# Autodesk Inventor assembly: MECANISMO DE COMPACTADO
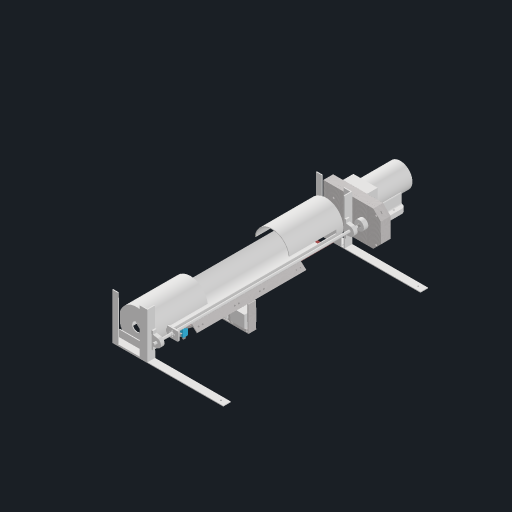
[picture p0: Inventor's stored thumbnail of the model, 512x512]
Saved by Autodesk Inventor 2024.3 (Build 283343000, 343)
## iProperties
Created: 2024-05-26
Part Number: MECANISMO DE COMPACTADO
Document SubType Name: Assembly
Designer: Jhuliams
Author: Jhuliams
## Documents named in this file (32)
- C:\Users\Niler\OneDrive\Escritorio\RECICLADOR\RECICLADOR_MODELO_3D\MECANISMO DE COMPACTADO\MECANISMO DE COMPACTADO.iam
- C:\Users\Niler\OneDrive\Escritorio\RECICLADOR\RECICLADOR_MODELO_3D\MECANISMO DE COMPACTADO\GUIA_DE_OBJETO.ipt
- C:\Users\Niler\OneDrive\Escritorio\RECICLADOR\RECICLADOR_MODELO_3D\MECANISMO DE COMPACTADO\TAPA QUE DESPLAZA CON TORNILLOS.ipt
- C:\Users\Niler\OneDrive\Escritorio\RECICLADOR\RECICLADOR_MODELO_3D\MECANISMO DE COMPACTADO\TUERCA DE HUSILLO.ipt
- C:\Users\Niler\OneDrive\Escritorio\RECICLADOR\RECICLADOR_MODELO_3D\MECANISMO DE COMPACTADO\TORNILLO DEPOTENCIA.ipt
- C:\Users\Niler\OneDrive\Escritorio\RECICLADOR\RECICLADOR_MODELO_3D\MECANISMO DE COMPACTADO\ACOPLE HELICOIDAL.ipt
- C:\Users\Niler\OneDrive\Escritorio\RECICLADOR\RECICLADOR_MODELO_3D\MECANISMO DE COMPACTADO\RODAMIENTO DE TORNILLO.ipt
- C:\Users\Niler\OneDrive\Escritorio\RECICLADOR\RECICLADOR_MODELO_3D\MECANISMO DE COMPACTADO\PLETINA PARA GUIA CILINDRICA.ipt
- C:\Users\Niler\OneDrive\Escritorio\RECICLADOR\RECICLADOR_MODELO_3D\MECANISMO DE COMPACTADO\SOPORTE LATERAL DE GUIA CILINDRICA.ipt
- C:\Users\Niler\OneDrive\Escritorio\RECICLADOR\RECICLADOR_MODELO_3D\MECANISMO DE COMPACTADO\SOPORTE LATERAL DE GUIA CILINDRICA_MIR.ipt
- C:\Users\Niler\OneDrive\Escritorio\RECICLADOR\RECICLADOR_MODELO_3D\MECANISMO DE COMPACTADO\RODAMIENTO DE TORNILLO_MIR.ipt
- C:\Users\Niler\OneDrive\Escritorio\RECICLADOR\RECICLADOR_MODELO_3D\MECANISMO DE COMPACTADO\SOPORTE LATERAL DE GUIA CILINDRICA_MIR1.ipt
- C:\Users\Niler\OneDrive\Escritorio\RECICLADOR\RECICLADOR_MODELO_3D\MECANISMO DE COMPACTADO\RODAMIENTO DE TORNILLO_MIR1.ipt
- C:\Users\Niler\OneDrive\Escritorio\RECICLADOR\RECICLADOR_MODELO_3D\MECANISMO DE COMPACTADO\SOPORTE LATERAL DE GUIA CILINDRICA_MIR2.ipt
- C:\Users\Niler\OneDrive\Escritorio\RECICLADOR\RECICLADOR_MODELO_3D\MECANISMO DE COMPACTADO\RODAMIENTO DE TORNILLO_MIR_MIR.ipt
- C:\Users\Niler\OneDrive\Escritorio\RECICLADOR\RECICLADOR_MODELO_3D\MECANISMO DE COMPACTADO\SOPORTE LATERAL DE GUIA CILINDRICA_MIR1_MIR.ipt
- C:\Users\Niler\OneDrive\Escritorio\RECICLADOR\RECICLADOR_MODELO_3D\MECANISMO DE COMPACTADO\ACOPLE HELICOIDAL_MIR.ipt
- C:\Users\Niler\OneDrive\Escritorio\RECICLADOR\RECICLADOR_MODELO_3D\CAJA_ENGRANAJES\VERSION_3\CAJA_ENGRANAJES_COMPLETA_V3.iam
- C:\Users\Niler\OneDrive\Escritorio\RECICLADOR\RECICLADOR_MODELO_3D\NUEVA_PARTE_MECANISMO_COMPACTADO\CANALETA_MOVIL.ipt
- C:\Users\Niler\OneDrive\Escritorio\RECICLADOR\RECICLADOR_MODELO_3D\NUEVA_PARTE_MECANISMO_COMPACTADO\APORYO_CANALETA_,MOVIL.ipt
- C:\Users\Niler\OneDrive\Escritorio\RECICLADOR\RECICLADOR_MODELO_3D\NUEVA_PARTE_MECANISMO_COMPACTADO\PLENTINA_CANALETA_MOVIL.ipt
- C:\Users\Niler\OneDrive\Escritorio\RECICLADOR\RECICLADOR_MODELO_3D\NUEVA_PARTE_MECANISMO_COMPACTADO\APORYO_CANALETA_,MOVIL_P2.ipt
- C:\Users\Niler\OneDrive\Escritorio\RECICLADOR\RECICLADOR_MODELO_3D\NUEVA_PARTE_MECANISMO_COMPACTADO\CREMALLERA_CANALETA_MOVIL.ipt
- C:\Users\Niler\OneDrive\Escritorio\RECICLADOR\RECICLADOR_MODELO_3D\NUEVA_PARTE_MECANISMO_COMPACTADO\SOPORTE_METAL_PAP.ipt
- C:\Users\Niler\OneDrive\Escritorio\RECICLADOR\RECICLADOR_MODELO_3D\MECANISMO DE COMPACTADO\PINON DE TAPA PRINCIPAL.ipt
- C:\Users\Niler\OneDrive\Escritorio\RECICLADOR\RECICLADOR_MODELO_3D\MECANISMO DE COMPACTADO\NEMA 17 PARA TAPA PRINCIPAL.ipt
- C:\Users\Niler\OneDrive\Escritorio\RECICLADOR\RECICLADOR_MODELO_3D\MECANISMO DE COMPACTADO\ACOPLE_NEMA_PUERTA.ipt
- C:\Users\Niler\OneDrive\Escritorio\RECICLADOR\RECICLADOR_MODELO_3D\VERSION_3_COMPLETA\FIN_DE_CARRERA.ipt
- C:\Users\Niler\OneDrive\Escritorio\RECICLADOR\RECICLADOR_MODELO_3D\NUEVA_PARTE_MECANISMO_COMPACTADO\APORYO_CANALETA_,MOVIL_MIR.ipt
- C:\Users\Niler\OneDrive\Escritorio\RECICLADOR\RECICLADOR_MODELO_3D\VERSION_3_COMPLETA\FIN_DE_CARRERA_MIR.ipt
- C:\Users\Niler\OneDrive\Escritorio\RECICLADOR\RECICLADOR_MODELO_3D\NUEVA_PARTE_MECANISMO_COMPACTADO\SOPORTE_CANALETA_PRINCIPAL.ipt
- C:\Users\Niler\OneDrive\Escritorio\RECICLADOR\RECICLADOR_MODELO_3D\Spur Gear11.ipt
## Components (39 placed, 31 different names)
1. PLETINA PARA GUIA CILINDRICA:1 — Mate:22, Flush:3, Mate:24, Flush:4, Flush:7, Flush:13, Flush:15, Mate:37
2. GUIA_DE_OBJETO:1 — Mate:6, Mate:7, Mate:8, Flush:2, Mate:21, Tangent:1, Mate:29, Tangent:2, Mate:42, Flush:23, Mate:52, Flush:25, Flush:30
3. TORNILLO DEPOTENCIA:1 — Mate:9, Mate:16, Flush:1, Mate:23, Mate:27, Flush:12, Mate:38, Mate:39
4. TORNILLO DEPOTENCIA:2 — Mate:10, Mate:15, Flush:1, Mate:34, Mate:35
5. TAPA QUE DESPLAZA CON TORNILLOS:1 — Mate:6, Mate:7, Mate:8, Mate:9, Mate:10, Mate:17, Mate:18, Mate:19, Mate:20
6. TUERCA DE HUSILLO:1 — Mate:16, Mate:17, Mate:20
7. TUERCA DE HUSILLO:2 — Mate:15, Mate:18, Mate:19
8. SOPORTE LATERAL DE GUIA CILINDRICA:1 — Flush:2, Mate:21, Tangent:1, Mate:22, Flush:3
9. SOPORTE LATERAL DE GUIA CILINDRICA_MIR:1 — Mate:29, Tangent:2, Mate:31, Flush:8, Mate:80
10. RODAMIENTO DE TORNILLO:1 — Mate:23, Mate:25, Flush:6, Flush:12
11. SOPORTE LATERAL DE GUIA CILINDRICA:2 — Mate:24, Mate:25, Flush:4, Flush:6
12. RODAMIENTO DE TORNILLO_MIR:1 — Mate:26, Flush:5, Mate:27
13. SOPORTE LATERAL DE GUIA CILINDRICA_MIR1:1 — Mate:26, Flush:5, Mate:30, Flush:9, Flush:22
14. PLETINA PARA GUIA CILINDRICA:2 — Flush:7, Mate:30, Mate:31, Flush:8, Flush:9, Flush:13, Mate:36, Flush:14, Flush:22
15. RODAMIENTO DE TORNILLO_MIR1:1 — Flush:10, Mate:32, Mate:35
16. SOPORTE LATERAL DE GUIA CILINDRICA_MIR2:1 — Flush:10, Mate:32, Flush:15, Mate:37
17. RODAMIENTO DE TORNILLO_MIR_MIR:1 — Flush:11, Mate:33, Mate:34
18. SOPORTE LATERAL DE GUIA CILINDRICA_MIR1_MIR:1 — Flush:11, Mate:33, Mate:36, Flush:14
19. ACOPLE HELICOIDAL:1 — Mate:38, Mate:39, Mate:40
20. ACOPLE HELICOIDAL_MIR:1 — Mate:41
21. CAJA_ENGRANAJES_COMPLETA_V3:1 [sub-assembly] — Mate:40, Mate:41
22. CANALETA_MOVIL:1 — Mate:42, Flush:23, Mate:65, Flush:26, Flush:27
23. APORYO_CANALETA_,MOVIL:1 — Mate:44, Mate:45, Mate:48, Mate:49, Mate:50, Mate:52, Mate:74, Mate:75, Mate:76, Flush:30
24. PLENTINA_CANALETA_MOVIL:1 — Mate:49, Mate:50, Mate:56, Mate:57, Mate:58, Mate:62, Mate:63, Mate:64, Mate:66
25. PLENTINA_CANALETA_MOVIL:2 — Mate:44, Mate:45, Mate:48, Flush:25, Mate:53, Mate:54, Mate:55, Mate:59, Mate:60, Mate:61, Mate:67, Flush:28
26. APORYO_CANALETA_,MOVIL_P2:1 — Mate:53, Mate:54, Mate:55
27. APORYO_CANALETA_,MOVIL_P2:2 — Mate:59, Mate:60, Mate:61
28. APORYO_CANALETA_,MOVIL_P2:3 — Mate:56, Mate:57, Mate:58
29. APORYO_CANALETA_,MOVIL_P2:4 — Mate:62, Mate:63, Mate:64
30. CREMALLERA_CANALETA_MOVIL:1 — Mate:65, Flush:26, Flush:27, Rotation/Translation:1
31. SOPORTE_METAL_PAP:1 — Mate:66, Mate:67, Flush:28, Mate:72, Flush:29, Mate:73
32. PINON DE TAPA PRINCIPAL:1 — Rotation/Translation:1, Mate:81, Mate:82
33. NEMA 17 PARA TAPA PRINCIPAL:1 — Mate:81
34. ACOPLE_NEMA_PUERTA:1 — Mate:72, Flush:29, Mate:73
35. FIN_DE_CARRERA:1 — Mate:74, Mate:75, Mate:76
36. APORYO_CANALETA_,MOVIL_MIR:1 — Mate:77, Mate:78, Mate:79
37. FIN_DE_CARRERA_MIR:1 — Mate:77, Mate:78, Mate:79
38. SOPORTE_CANALETA_PRINCIPAL:1 — Mate:80
39. Spur Gear1:1 — Mate:82
## Relationships (95: Mate 68, Flush 23, Tangent 2, Angle 1, RelateRotateTranslate 1)
- Mate:6: GUIA_DE_OBJETO:1 ↔ TAPA QUE DESPLAZA CON TORNILLOS:1
- Mate:7 (1 mm): GUIA_DE_OBJETO:1 ↔ TAPA QUE DESPLAZA CON TORNILLOS:1
- Mate:8 (1 mm): GUIA_DE_OBJETO:1 ↔ TAPA QUE DESPLAZA CON TORNILLOS:1
- Mate:9: TORNILLO DEPOTENCIA:1 ↔ TAPA QUE DESPLAZA CON TORNILLOS:1
- Mate:10: TORNILLO DEPOTENCIA:2 ↔ TAPA QUE DESPLAZA CON TORNILLOS:1
- Mate:15: TORNILLO DEPOTENCIA:2 ↔ TUERCA DE HUSILLO:2
- Mate:16: TORNILLO DEPOTENCIA:1 ↔ TUERCA DE HUSILLO:1
- Mate:17: TAPA QUE DESPLAZA CON TORNILLOS:1 ↔ TUERCA DE HUSILLO:1
- Mate:18: TAPA QUE DESPLAZA CON TORNILLOS:1 ↔ TUERCA DE HUSILLO:2
- Mate:19: TAPA QUE DESPLAZA CON TORNILLOS:1 ↔ TUERCA DE HUSILLO:2
- Mate:20: TAPA QUE DESPLAZA CON TORNILLOS:1 ↔ TUERCA DE HUSILLO:1
- Flush:1: TORNILLO DEPOTENCIA:1 ↔ TORNILLO DEPOTENCIA:2
- Flush:2 (48.325 mm): GUIA_DE_OBJETO:1 ↔ SOPORTE LATERAL DE GUIA CILINDRICA:1
- Mate:21: GUIA_DE_OBJETO:1 ↔ SOPORTE LATERAL DE GUIA CILINDRICA:1
- Tangent:1 (-7.5 mm): GUIA_DE_OBJETO:1 ↔ SOPORTE LATERAL DE GUIA CILINDRICA:1
- Mate:22: PLETINA PARA GUIA CILINDRICA:1 ↔ SOPORTE LATERAL DE GUIA CILINDRICA:1
- Flush:3: PLETINA PARA GUIA CILINDRICA:1 ↔ SOPORTE LATERAL DE GUIA CILINDRICA:1
- Mate:23: TORNILLO DEPOTENCIA:1 ↔ RODAMIENTO DE TORNILLO:1
- Mate:24: PLETINA PARA GUIA CILINDRICA:1 ↔ SOPORTE LATERAL DE GUIA CILINDRICA:2
- Mate:25: RODAMIENTO DE TORNILLO:1 ↔ SOPORTE LATERAL DE GUIA CILINDRICA:2
- Flush:4: PLETINA PARA GUIA CILINDRICA:1 ↔ SOPORTE LATERAL DE GUIA CILINDRICA:2
- Mate:26: RODAMIENTO DE TORNILLO_MIR:1 ↔ SOPORTE LATERAL DE GUIA CILINDRICA_MIR1:1
- Flush:5: RODAMIENTO DE TORNILLO_MIR:1 ↔ SOPORTE LATERAL DE GUIA CILINDRICA_MIR1:1
- Mate:27: TORNILLO DEPOTENCIA:1 ↔ RODAMIENTO DE TORNILLO_MIR:1
- Flush:6: RODAMIENTO DE TORNILLO:1 ↔ SOPORTE LATERAL DE GUIA CILINDRICA:2
- Mate:29: GUIA_DE_OBJETO:1 ↔ SOPORTE LATERAL DE GUIA CILINDRICA_MIR:1
- Tangent:2 (-107.5 mm): GUIA_DE_OBJETO:1 ↔ SOPORTE LATERAL DE GUIA CILINDRICA_MIR:1
- Flush:7: PLETINA PARA GUIA CILINDRICA:1 ↔ PLETINA PARA GUIA CILINDRICA:2
- Mate:30: SOPORTE LATERAL DE GUIA CILINDRICA_MIR1:1 ↔ PLETINA PARA GUIA CILINDRICA:2
- Mate:31: SOPORTE LATERAL DE GUIA CILINDRICA_MIR:1 ↔ PLETINA PARA GUIA CILINDRICA:2
- Flush:8: SOPORTE LATERAL DE GUIA CILINDRICA_MIR:1 ↔ PLETINA PARA GUIA CILINDRICA:2
- Flush:9: SOPORTE LATERAL DE GUIA CILINDRICA_MIR1:1 ↔ PLETINA PARA GUIA CILINDRICA:2
- Flush:10: RODAMIENTO DE TORNILLO_MIR1:1 ↔ SOPORTE LATERAL DE GUIA CILINDRICA_MIR2:1
- Mate:32: RODAMIENTO DE TORNILLO_MIR1:1 ↔ SOPORTE LATERAL DE GUIA CILINDRICA_MIR2:1
- Flush:11: RODAMIENTO DE TORNILLO_MIR_MIR:1 ↔ SOPORTE LATERAL DE GUIA CILINDRICA_MIR1_MIR:1
- Mate:33: RODAMIENTO DE TORNILLO_MIR_MIR:1 ↔ SOPORTE LATERAL DE GUIA CILINDRICA_MIR1_MIR:1
- Flush:12 (10 mm): TORNILLO DEPOTENCIA:1 ↔ RODAMIENTO DE TORNILLO:1
- Flush:13: PLETINA PARA GUIA CILINDRICA:1 ↔ PLETINA PARA GUIA CILINDRICA:2
- Mate:34: TORNILLO DEPOTENCIA:2 ↔ RODAMIENTO DE TORNILLO_MIR_MIR:1
- Mate:35: TORNILLO DEPOTENCIA:2 ↔ RODAMIENTO DE TORNILLO_MIR1:1
- Mate:36: PLETINA PARA GUIA CILINDRICA:2 ↔ SOPORTE LATERAL DE GUIA CILINDRICA_MIR1_MIR:1
- Flush:14: PLETINA PARA GUIA CILINDRICA:2 ↔ SOPORTE LATERAL DE GUIA CILINDRICA_MIR1_MIR:1
- Flush:15: PLETINA PARA GUIA CILINDRICA:1 ↔ SOPORTE LATERAL DE GUIA CILINDRICA_MIR2:1
- Mate:37: PLETINA PARA GUIA CILINDRICA:1 ↔ SOPORTE LATERAL DE GUIA CILINDRICA_MIR2:1
- Mate:38 (-20 mm): TORNILLO DEPOTENCIA:1 ↔ ACOPLE HELICOIDAL:1
- Mate:39: TORNILLO DEPOTENCIA:1 ↔ ACOPLE HELICOIDAL:1
- Flush:22 (250 mm): SOPORTE LATERAL DE GUIA CILINDRICA_MIR1:1 ↔ PLETINA PARA GUIA CILINDRICA:2
- Mate:40: ACOPLE HELICOIDAL:1 ↔ CAJA_ENGRANAJES_COMPLETA_V3:1
- Mate:41: ACOPLE HELICOIDAL_MIR:1 ↔ CAJA_ENGRANAJES_COMPLETA_V3:1
- Mate:42: GUIA_DE_OBJETO:1 ↔ CANALETA_MOVIL:1
- Flush:23: GUIA_DE_OBJETO:1 ↔ CANALETA_MOVIL:1
- Mate:44: APORYO_CANALETA_,MOVIL:1 ↔ PLENTINA_CANALETA_MOVIL:2
- Mate:45: APORYO_CANALETA_,MOVIL:1 ↔ PLENTINA_CANALETA_MOVIL:2
- Mate:48: APORYO_CANALETA_,MOVIL:1 ↔ PLENTINA_CANALETA_MOVIL:2
- Mate:49: APORYO_CANALETA_,MOVIL:1 ↔ PLENTINA_CANALETA_MOVIL:1
- Mate:50: APORYO_CANALETA_,MOVIL:1 ↔ PLENTINA_CANALETA_MOVIL:1
- Mate:52: GUIA_DE_OBJETO:1 ↔ APORYO_CANALETA_,MOVIL:1
- Flush:25: GUIA_DE_OBJETO:1 ↔ PLENTINA_CANALETA_MOVIL:2
- Mate:53: PLENTINA_CANALETA_MOVIL:2 ↔ APORYO_CANALETA_,MOVIL_P2:1
- Mate:54: PLENTINA_CANALETA_MOVIL:2 ↔ APORYO_CANALETA_,MOVIL_P2:1
- Mate:55: PLENTINA_CANALETA_MOVIL:2 ↔ APORYO_CANALETA_,MOVIL_P2:1
- Mate:56: PLENTINA_CANALETA_MOVIL:1 ↔ APORYO_CANALETA_,MOVIL_P2:3
- Mate:57: PLENTINA_CANALETA_MOVIL:1 ↔ APORYO_CANALETA_,MOVIL_P2:3
- Mate:58: PLENTINA_CANALETA_MOVIL:1 ↔ APORYO_CANALETA_,MOVIL_P2:3
- Mate:59: PLENTINA_CANALETA_MOVIL:2 ↔ APORYO_CANALETA_,MOVIL_P2:2
- Mate:60: PLENTINA_CANALETA_MOVIL:2 ↔ APORYO_CANALETA_,MOVIL_P2:2
- Mate:61: PLENTINA_CANALETA_MOVIL:2 ↔ APORYO_CANALETA_,MOVIL_P2:2
- Mate:62: PLENTINA_CANALETA_MOVIL:1 ↔ APORYO_CANALETA_,MOVIL_P2:4
- Mate:63: PLENTINA_CANALETA_MOVIL:1 ↔ APORYO_CANALETA_,MOVIL_P2:4
- Mate:64: PLENTINA_CANALETA_MOVIL:1 ↔ APORYO_CANALETA_,MOVIL_P2:4
- Mate:65: CANALETA_MOVIL:1 ↔ CREMALLERA_CANALETA_MOVIL:1
- Flush:26: CANALETA_MOVIL:1 ↔ CREMALLERA_CANALETA_MOVIL:1
- Flush:27: CANALETA_MOVIL:1 ↔ CREMALLERA_CANALETA_MOVIL:1
- Mate:66: PLENTINA_CANALETA_MOVIL:1 ↔ SOPORTE_METAL_PAP:1
- Mate:67: PLENTINA_CANALETA_MOVIL:2 ↔ SOPORTE_METAL_PAP:1
- [Mate]: PINON DE TAPA PRINCIPAL:1 ↔ NEMA 17 PARA TAPA PRINCIPAL:1
- [Mate] (10 mm): PINON DE TAPA PRINCIPAL:1 ↔ NEMA 17 PARA TAPA PRINCIPAL:1
- [Mate]: NEMA 17 PARA TAPA PRINCIPAL:1 ↔ ACOPLE_NEMA_PUERTA:1
- [Mate]: NEMA 17 PARA TAPA PRINCIPAL:1 ↔ ACOPLE_NEMA_PUERTA:1
- [Angle] (0 deg): NEMA 17 PARA TAPA PRINCIPAL:1 ↔ ACOPLE_NEMA_PUERTA:1
- Flush:28: PLENTINA_CANALETA_MOVIL:2 ↔ SOPORTE_METAL_PAP:1
- Mate:72: SOPORTE_METAL_PAP:1 ↔ ACOPLE_NEMA_PUERTA:1
- Flush:29: SOPORTE_METAL_PAP:1 ↔ ACOPLE_NEMA_PUERTA:1
- Mate:73: SOPORTE_METAL_PAP:1 ↔ ACOPLE_NEMA_PUERTA:1
- Mate:74: APORYO_CANALETA_,MOVIL:1 ↔ FIN_DE_CARRERA:1
- Mate:75: APORYO_CANALETA_,MOVIL:1 ↔ FIN_DE_CARRERA:1
- Mate:76: APORYO_CANALETA_,MOVIL:1 ↔ FIN_DE_CARRERA:1
- Flush:30: GUIA_DE_OBJETO:1 ↔ APORYO_CANALETA_,MOVIL:1
- Mate:77: APORYO_CANALETA_,MOVIL_MIR:1 ↔ FIN_DE_CARRERA_MIR:1
- Mate:78: APORYO_CANALETA_,MOVIL_MIR:1 ↔ FIN_DE_CARRERA_MIR:1
- Mate:79: APORYO_CANALETA_,MOVIL_MIR:1 ↔ FIN_DE_CARRERA_MIR:1
- Rotation/Translation:1 [RelateRotateTranslate] (169 mm): CREMALLERA_CANALETA_MOVIL:1 ↔ PINON DE TAPA PRINCIPAL:1
- Mate:80: SOPORTE LATERAL DE GUIA CILINDRICA_MIR:1 ↔ SOPORTE_CANALETA_PRINCIPAL:1
- Mate:81: PINON DE TAPA PRINCIPAL:1 ↔ NEMA 17 PARA TAPA PRINCIPAL:1
- Mate:82: PINON DE TAPA PRINCIPAL:1 ↔ Spur Gear1:1
